# Autodesk Inventor assembly: Captador Assembly
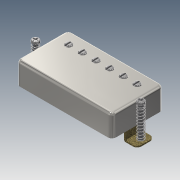
[picture p0: Inventor's stored thumbnail of the model, 180x180]
Saved by Autodesk Inventor 2016 (Build 200138000, 138)
## iProperties
Created: 2018-12-12
Part Number: Captador Assembly
Document SubType Name: Assembly
Designer: Pedro Mendonça
Author: Pedro Mendonça
## Documents named in this file (5)
- C:\Users\Pedro\Google Drive\Projeto CAD Eng Mecânica\Captador Assembly.iam
- C:\Users\Pedro\Google Drive\Projeto CAD Eng Mecânica\captador- Lesly.ipt
- C:\Users\Pedro\Google Drive\Projeto CAD Eng Mecânica\parafuso do captador( necessita de reparo).ipt
- C:\Users\Pedro\Google Drive\Projeto CAD Eng Mecânica\Parafuso lateral do captador.ipt
- C:\Users\Pedro\Google Drive\Projeto CAD Eng Mecânica\Mola do Captador.ipt
## Components (11 placed, 4 different names)
1. captador- Lesly:2 — Insert:1, Insert:2, Insert:3, Insert:4, Insert:5, Insert:6, Insert:7, Insert:8
2. parafuso do captador( necessita de reparo):1 — Insert:1
3. parafuso do captador( necessita de reparo):2 — Insert:2
4. parafuso do captador( necessita de reparo):3 — Insert:3
5. parafuso do captador( necessita de reparo):4 — Insert:4
6. parafuso do captador( necessita de reparo):5 — Insert:5
7. parafuso do captador( necessita de reparo):6 — Insert:6
8. Parafuso lateral do captador:1 — Insert:8
9. Parafuso lateral do captador:2 — Insert:7
10. Mola do Captador:1
11. Mola do Captador:2
## Relationships (8: Insert 8)
- Insert:1 (1 mm): captador- Lesly:2 ↔ parafuso do captador( necessita de reparo):1
- Insert:2 (1 mm): captador- Lesly:2 ↔ parafuso do captador( necessita de reparo):2
- Insert:3 (1 mm): captador- Lesly:2 ↔ parafuso do captador( necessita de reparo):3
- Insert:4 (1 mm): captador- Lesly:2 ↔ parafuso do captador( necessita de reparo):4
- Insert:5 (1 mm): captador- Lesly:2 ↔ parafuso do captador( necessita de reparo):5
- Insert:6 (1 mm): captador- Lesly:2 ↔ parafuso do captador( necessita de reparo):6
- Insert:7: captador- Lesly:2 ↔ Parafuso lateral do captador:2
- Insert:8: captador- Lesly:2 ↔ Parafuso lateral do captador:1
